# Autodesk Inventor assembly: Piston Bracket Assembly - L
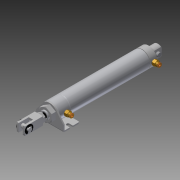
[picture p0: Inventor's stored thumbnail of the model, 180x180]
Saved by Autodesk Inventor 2014 SP1 (Build 180222100, 222)
## iProperties
Created: 2013-03-16
Part Number: Piston Bracket Assembly - L
Document SubType Name: Assembly
Designer: Arpan
Mass: 1128.04 g
Surface Area: 993.127 cm^2
Volume: 159.546 cm^3
Density: 7.07031 g/cm^3
Author: Arpan
## Documents named in this file (4)
- C:\Users\Moses\Documents\Inventor\Sally Rebuild\Rebuild Sally\Piston Bracket Assembly - L.iam
- C:\Users\Moses\Documents\Inventor\Sally Rebuild\Rebuild Sally\ninja cylinder foot bracket.ipt
- C:\Users\Moses\Documents\Inventor\Sally Rebuild\Rebuild Sally\Pneumatics\Pneumatics_SMC_KQ2H03-34S.ipt
- C:\Users\Moses\Documents\Inventor\Sally Rebuild\Rebuild Sally\Rebuild good piston - L.iam
## Components (4 placed, 3 different names)
1. ninja cylinder foot bracket:1 — Mate:1, Mate:2, Angle:1
2. Rebuild good piston - L:1 [sub-assembly] — Mate:1, Mate:2, Angle:1, Insert:1, Insert:2
3. Pneumatics_SMC_KQ2H03-34S:1 — Insert:1
4. Pneumatics_SMC_KQ2H03-34S:2 — Insert:2
## Relationships (5: Mate 2, Insert 2, Angle 1)
- Mate:1: ninja cylinder foot bracket:1 ↔ Rebuild good piston - L:1
- Mate:2: ninja cylinder foot bracket:1 ↔ Rebuild good piston - L:1
- Angle:1 (0 deg): ninja cylinder foot bracket:1 ↔ Rebuild good piston - L:1
- Insert:1 (1.27 mm): Rebuild good piston - L:1 ↔ Pneumatics_SMC_KQ2H03-34S:1
- Insert:2 (1.27 mm): Rebuild good piston - L:1 ↔ Pneumatics_SMC_KQ2H03-34S:2
